# Autodesk Inventor assembly: Full Large Bearing
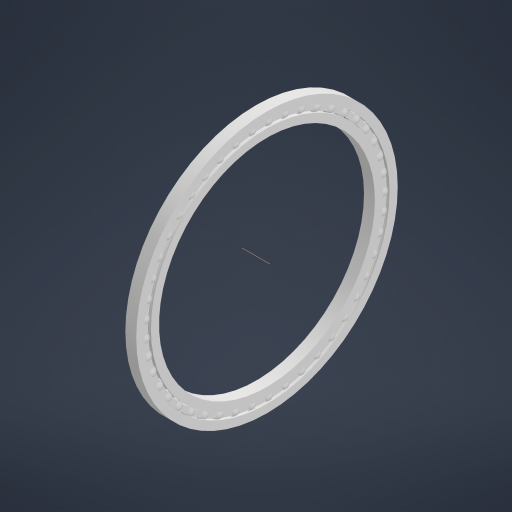
[picture p0: Inventor's stored thumbnail of the model, 512x512]
Saved by Autodesk Inventor 2023 (Build 270158000, 158)
## iProperties
Created: 2022-11-20
Part Number: Full Large Bearing
Document SubType Name: Assembly
Designer: Izack Waczko
Author: Izack Waczko
## Documents named in this file (3)
- D:\CAD Modeling\Private Robotics\Custom Tryhard Robot\Drivetrain\Swerve Module Parts\Bearing Parts\Full Large Bearing.iam
- D:\CAD Modeling\Private Robotics\Custom Tryhard Robot\Drivetrain\Swerve Module Parts\Bearing Parts\Large bearing.ipt
- D:\CAD Modeling\Private Robotics\Custom Tryhard Robot\Drivetrain\Swerve Module Parts\Bearing Parts\Large Bearing Spacer.ipt
## Components (2 placed, 2 different names)
1. Large bearing:1 — Mate:1, Flush:1, Mate:2
2. Large Bearing Spacer:1 — Flush:1, Mate:2
## Relationships (3: Mate 2, Flush 1)
- Mate:1: Large bearing:1
- Flush:1: Large bearing:1 ↔ Large Bearing Spacer:1
- Mate:2: Large bearing:1 ↔ Large Bearing Spacer:1
